# Autodesk Inventor assembly: Filament_dryer
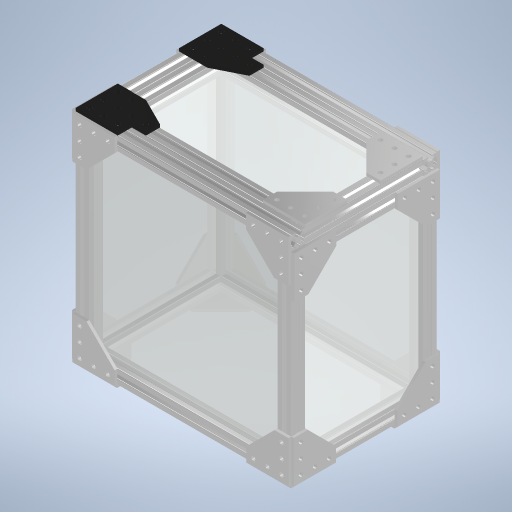
[picture p0: Inventor's stored thumbnail of the model, 512x512]
Saved by Autodesk Inventor 2024 (Build 280153000, 153)
## iProperties
Created: 2024-09-20
Part Number: Filament_dryer
Document SubType Name: Assembly
Designer: Owner
Author: Owner
## Documents named in this file (12)
- C:\Users\Owner\Desktop\Work\Filament dryer\Filament_dryer.iam
- C:\Users\Owner\Desktop\Work\Filament dryer\panel_14x9.ipt
- C:\Users\Owner\Desktop\Work\Filament dryer\T_slot_1in_8.35in.ipt
- C:\Users\Owner\Desktop\Work\Filament dryer\T_slot_1in_15.35in.ipt
- C:\Users\Owner\Desktop\Work\Filament dryer\panel_14x14.ipt
- C:\Users\Owner\Desktop\Work\Filament dryer\T_slot_1in_13.35in.ipt
- C:\Users\Owner\Desktop\Work\Filament dryer\panel_13x7.ipt
- C:\Users\Owner\Desktop\Work\Filament dryer\T_slot_1in_12.35in.ipt
- C:\Users\Owner\Desktop\Work\Filament dryer\panel_13x9.ipt
- C:\Users\Owner\Desktop\Work\Filament dryer\corner_bracket.ipt
- C:\Users\Owner\Desktop\Work\Filament dryer\47065T267_T-Slotted Framing_cut.ipt
- C:\Users\Owner\Desktop\Work\Filament dryer\corner_bracket_flush.ipt
## Components (48 placed, 11 different names)
1. panel_14x9:1 — Mate:1, Tangent:1, Flush:1, Mate:2, Flush:2, Tangent:2, Mate:3, Mate:4
2. T_slot_1in_8.35in:1 — Mate:2, Flush:2, Tangent:2, Mate:17, Flush:58, Flush:61, Flush:67, Flush:69
3. T_slot_1in_8.35in:2 — Mate:1, Tangent:1, Flush:1, Flush:3, Flush:4, Flush:5, Flush:6, Mate:32, Mate:40, Flush:35, Flush:36, Flush:63, Flush:64
4. T_slot_1in_15.35in:1 — Mate:3, Flush:3, Flush:4, Mate:5, Tangent:3, Flush:7, Mate:10, Mate:38, Flush:31, Mate:39, Flush:33, Mate:52, Mate:55, Flush:65, Mate:57, Flush:68
5. T_slot_1in_15.35in:2 — Mate:4, Flush:5, Flush:6, Mate:6, Tangent:4, Flush:8, Mate:12, Mate:16, Mate:41, Mate:50, Flush:54, Mate:51, Flush:57, Mate:53, Mate:54, Flush:62, Mate:56, Flush:66
6. panel_14x14:1 — Mate:5, Tangent:3, Flush:7, Mate:7, Tangent:5, Flush:9, Mate:9, Mate:13
7. panel_14x14:2 — Mate:6, Tangent:4, Flush:8, Mate:8, Tangent:6, Flush:10, Mate:11, Mate:15
8. T_slot_1in_15.35in:3 — Mate:8, Tangent:6, Flush:10, Flush:12, Flush:14, Mate:20, Flush:15, Mate:24, Mate:29, Flush:21, Flush:38, Mate:48, Mate:49, Flush:52, Flush:75
9. T_slot_1in_15.35in:4 — Mate:7, Tangent:5, Flush:9, Flush:11, Mate:14, Flush:13, Mate:23, Flush:18, Mate:27, Flush:20, Mate:34, Flush:22, Mate:35, Flush:24, Flush:25, Mate:47, Mate:61, Flush:77
10. T_slot_1in_13.35in:1 — Mate:15, Flush:14, Mate:16, Mate:21, Flush:16, Flush:17, Mate:33, Tangent:9, Mate:37, Flush:29, Flush:37, Mate:42, Flush:39, Flush:56
11. T_slot_1in_13.35in:2 — Mate:13, Mate:14, Flush:13, Mate:36, Flush:26, Flush:32, Flush:34
12. T_slot_1in_13.35in:3 — Mate:11, Flush:12, Mate:12, Flush:51, Flush:53, Flush:55, Flush:60
13. T_slot_1in_13.35in:4 — Mate:9, Flush:11, Mate:10, Mate:18, Tangent:7, Flush:23, Flush:30, Flush:49, Flush:59
14. panel_14x9:2 — Mate:17, Mate:18, Tangent:7, Mate:19
15. T_slot_1in_8.35in:3 — Mate:19, Mate:20, Flush:15, Flush:19, Mate:25, Flush:48, Flush:50, Mate:60, Flush:74, Flush:76
16. T_slot_1in_8.35in:4 — Mate:22, Mate:23, Flush:18, Mate:43, Flush:41, Mate:44, Flush:43
17. T_slot_1in_8.35in:5 — Mate:21, Flush:16, Flush:17, Mate:22, Flush:27, Flush:28
18. T_slot_1in_8.35in:6 — Mate:24, Flush:19, Mate:25, Mate:26, Mate:28, Mate:30, Flush:71, Mate:59, Flush:73
19. T_slot_1in_12.35in:1 — Mate:28, Mate:29, Flush:21, Mate:31, Tangent:8, Flush:42, Flush:72
20. T_slot_1in_12.35in:2 — Mate:26, Mate:27, Flush:20, Flush:40, Mate:58, Flush:70
21. panel_13x7:1 — Mate:30, Mate:31, Tangent:8
22. panel_13x9:1 — Mate:32, Mate:33, Tangent:9
23. corner_bracket:1 — Mate:39, Flush:32, Flush:33
24. corner_bracket:2 — Mate:40, Flush:34, Flush:35
25. corner_bracket:3 — Mate:42, Flush:38, Flush:39
26. corner_bracket:4 — Mate:43, Flush:40, Flush:41
27. corner_bracket:5 — Mate:38, Flush:30, Flush:31
28. corner_bracket:6 — Mate:34, Flush:22, Flush:23
29. corner_bracket:7 — Mate:41, Flush:36, Flush:37
30. corner_bracket:8 — Mate:35, Flush:24, Flush:25
31. corner_bracket:9 — Mate:37, Flush:28, Flush:29
32. corner_bracket:10 — Mate:36, Flush:26, Flush:27
33. corner_bracket:11 — Mate:51, Flush:56, Flush:57
34. corner_bracket:12 — Mate:44, Flush:42, Flush:43
35. corner_bracket:14 — Mate:52, Flush:58, Flush:59
36. corner_bracket:15 — Mate:53, Flush:60, Flush:61
37. corner_bracket:16 — Mate:48, Flush:50, Flush:51
38. corner_bracket:18 — Mate:50, Flush:54, Flush:55
39. corner_bracket:19 — Mate:49, Flush:52, Flush:53
40. corner_bracket:20 — Mate:47, Flush:48, Flush:49
41. corner_bracket:21 — Mate:55, Flush:64, Flush:65
42. corner_bracket:22 — Mate:57, Flush:68, Flush:69
43. corner_bracket:23 — Mate:56, Flush:66, Flush:67
44. corner_bracket:24 — Mate:54, Flush:62, Flush:63
45. 47065T267_T-Slotted Framing_cut:1 — Mate:59, Flush:72, Flush:73
46. 47065T267_T-Slotted Framing_cut:2 — Mate:58, Flush:70, Flush:71
47. corner_bracket_flush:1 — Mate:60, Flush:74, Flush:75
48. corner_bracket_flush:2 — Mate:61, Flush:76, Flush:77
## Relationships (141: Flush 73, Mate 59, Tangent 9)
- Mate:1: panel_14x9:1 ↔ T_slot_1in_8.35in:2
- Tangent:1: panel_14x9:1 ↔ T_slot_1in_8.35in:2
- Flush:1 (8.255 mm): panel_14x9:1 ↔ T_slot_1in_8.35in:2
- Mate:2: panel_14x9:1 ↔ T_slot_1in_8.35in:1
- Flush:2 (8.255 mm): panel_14x9:1 ↔ T_slot_1in_8.35in:1
- Tangent:2: panel_14x9:1 ↔ T_slot_1in_8.35in:1
- Mate:3: panel_14x9:1 ↔ T_slot_1in_15.35in:1
- Flush:3: T_slot_1in_8.35in:2 ↔ T_slot_1in_15.35in:1
- Flush:4: T_slot_1in_8.35in:2 ↔ T_slot_1in_15.35in:1
- Mate:4: panel_14x9:1 ↔ T_slot_1in_15.35in:2
- Flush:5: T_slot_1in_8.35in:2 ↔ T_slot_1in_15.35in:2
- Flush:6: T_slot_1in_8.35in:2 ↔ T_slot_1in_15.35in:2
- Mate:5: T_slot_1in_15.35in:1 ↔ panel_14x14:1
- Tangent:3: T_slot_1in_15.35in:1 ↔ panel_14x14:1
- Flush:7 (16.51 mm): T_slot_1in_15.35in:1 ↔ panel_14x14:1
- Mate:6: T_slot_1in_15.35in:2 ↔ panel_14x14:2
- Tangent:4: T_slot_1in_15.35in:2 ↔ panel_14x14:2
- Flush:8 (16.51 mm): T_slot_1in_15.35in:2 ↔ panel_14x14:2
- Mate:7: panel_14x14:1 ↔ T_slot_1in_15.35in:4
- Tangent:5: panel_14x14:1 ↔ T_slot_1in_15.35in:4
- Flush:9 (-16.51 mm): panel_14x14:1 ↔ T_slot_1in_15.35in:4
- Mate:8: panel_14x14:2 ↔ T_slot_1in_15.35in:3
- Tangent:6: panel_14x14:2 ↔ T_slot_1in_15.35in:3
- Flush:10 (-16.51 mm): panel_14x14:2 ↔ T_slot_1in_15.35in:3
- Mate:9: panel_14x14:1 ↔ T_slot_1in_13.35in:4
- Flush:11: T_slot_1in_15.35in:4 ↔ T_slot_1in_13.35in:4
- Mate:10: T_slot_1in_15.35in:1 ↔ T_slot_1in_13.35in:4
- Mate:11: panel_14x14:2 ↔ T_slot_1in_13.35in:3
- Flush:12: T_slot_1in_15.35in:3 ↔ T_slot_1in_13.35in:3
- Mate:12: T_slot_1in_15.35in:2 ↔ T_slot_1in_13.35in:3
- Mate:13: panel_14x14:1 ↔ T_slot_1in_13.35in:2
- Mate:14: T_slot_1in_15.35in:4 ↔ T_slot_1in_13.35in:2
- Flush:13: T_slot_1in_15.35in:4 ↔ T_slot_1in_13.35in:2
- Mate:15: panel_14x14:2 ↔ T_slot_1in_13.35in:1
- Flush:14: T_slot_1in_15.35in:3 ↔ T_slot_1in_13.35in:1
- Mate:16: T_slot_1in_15.35in:2 ↔ T_slot_1in_13.35in:1
- Mate:17: T_slot_1in_8.35in:1 ↔ panel_14x9:2
- Mate:18: T_slot_1in_13.35in:4 ↔ panel_14x9:2
- Tangent:7: T_slot_1in_13.35in:4 ↔ panel_14x9:2
- Mate:19: panel_14x9:2 ↔ T_slot_1in_8.35in:3
- Mate:20: T_slot_1in_15.35in:3 ↔ T_slot_1in_8.35in:3
- Flush:15: T_slot_1in_15.35in:3 ↔ T_slot_1in_8.35in:3
- Mate:21: T_slot_1in_13.35in:1 ↔ T_slot_1in_8.35in:5
- Flush:16: T_slot_1in_13.35in:1 ↔ T_slot_1in_8.35in:5
- Flush:17: T_slot_1in_13.35in:1 ↔ T_slot_1in_8.35in:5
- Mate:22: T_slot_1in_8.35in:4 ↔ T_slot_1in_8.35in:5
- Mate:23: T_slot_1in_15.35in:4 ↔ T_slot_1in_8.35in:4
- Flush:18: T_slot_1in_15.35in:4 ↔ T_slot_1in_8.35in:4
- Mate:24: T_slot_1in_15.35in:3 ↔ T_slot_1in_8.35in:6
- Flush:19: T_slot_1in_8.35in:3 ↔ T_slot_1in_8.35in:6
- Mate:25: T_slot_1in_8.35in:3 ↔ T_slot_1in_8.35in:6
- Mate:26: T_slot_1in_8.35in:6 ↔ T_slot_1in_12.35in:2
- Mate:27: T_slot_1in_15.35in:4 ↔ T_slot_1in_12.35in:2
- Flush:20: T_slot_1in_15.35in:4 ↔ T_slot_1in_12.35in:2
- Mate:28: T_slot_1in_8.35in:6 ↔ T_slot_1in_12.35in:1
- Mate:29: T_slot_1in_15.35in:3 ↔ T_slot_1in_12.35in:1
- Flush:21: T_slot_1in_15.35in:3 ↔ T_slot_1in_12.35in:1
- Mate:30: T_slot_1in_8.35in:6 ↔ panel_13x7:1
- Mate:31: T_slot_1in_12.35in:1 ↔ panel_13x7:1
- Tangent:8: T_slot_1in_12.35in:1 ↔ panel_13x7:1
- Mate:32: T_slot_1in_8.35in:2 ↔ panel_13x9:1
- Mate:33: T_slot_1in_13.35in:1 ↔ panel_13x9:1
- Tangent:9: T_slot_1in_13.35in:1 ↔ panel_13x9:1
- Mate:34: T_slot_1in_15.35in:4 ↔ corner_bracket:6
- Flush:22: T_slot_1in_15.35in:4 ↔ corner_bracket:6
- Flush:23: T_slot_1in_13.35in:4 ↔ corner_bracket:6
- Mate:35: T_slot_1in_15.35in:4 ↔ corner_bracket:8
- Flush:24: T_slot_1in_15.35in:4 ↔ corner_bracket:8
- Flush:25: T_slot_1in_15.35in:4 ↔ corner_bracket:8
- Mate:36: T_slot_1in_13.35in:2 ↔ corner_bracket:10
- Flush:26: T_slot_1in_13.35in:2 ↔ corner_bracket:10
- Flush:27: T_slot_1in_8.35in:5 ↔ corner_bracket:10
- Mate:37: T_slot_1in_13.35in:1 ↔ corner_bracket:9
- Flush:28: T_slot_1in_8.35in:5 ↔ corner_bracket:9
- Flush:29: T_slot_1in_13.35in:1 ↔ corner_bracket:9
- Mate:38: T_slot_1in_15.35in:1 ↔ corner_bracket:5
- Flush:30: T_slot_1in_13.35in:4 ↔ corner_bracket:5
- Flush:31: T_slot_1in_15.35in:1 ↔ corner_bracket:5
- Mate:39: T_slot_1in_15.35in:1 ↔ corner_bracket:1
- Flush:32: T_slot_1in_13.35in:2 ↔ corner_bracket:1
- Flush:33: T_slot_1in_15.35in:1 ↔ corner_bracket:1
- Mate:40: T_slot_1in_8.35in:2 ↔ corner_bracket:2
- Flush:34: T_slot_1in_13.35in:2 ↔ corner_bracket:2
- Flush:35: T_slot_1in_8.35in:2 ↔ corner_bracket:2
- Mate:41: T_slot_1in_15.35in:2 ↔ corner_bracket:7
- Flush:36: T_slot_1in_8.35in:2 ↔ corner_bracket:7
- Flush:37: T_slot_1in_13.35in:1 ↔ corner_bracket:7
- Mate:42: T_slot_1in_13.35in:1 ↔ corner_bracket:3
- Flush:38: T_slot_1in_15.35in:3 ↔ corner_bracket:3
- Flush:39: T_slot_1in_13.35in:1 ↔ corner_bracket:3
- Mate:43: T_slot_1in_8.35in:4 ↔ corner_bracket:4
- Flush:40: T_slot_1in_12.35in:2 ↔ corner_bracket:4
- Flush:41: T_slot_1in_8.35in:4 ↔ corner_bracket:4
- Mate:44: T_slot_1in_8.35in:4 ↔ corner_bracket:12
- Flush:42: T_slot_1in_12.35in:1 ↔ corner_bracket:12
- Flush:43: T_slot_1in_8.35in:4 ↔ corner_bracket:12
- Mate:47: T_slot_1in_15.35in:4 ↔ corner_bracket:20
- Flush:48: T_slot_1in_8.35in:3 ↔ corner_bracket:20
- Flush:49: T_slot_1in_13.35in:4 ↔ corner_bracket:20
- Mate:48: T_slot_1in_15.35in:3 ↔ corner_bracket:16
- Flush:50: T_slot_1in_8.35in:3 ↔ corner_bracket:16
- Flush:51: T_slot_1in_13.35in:3 ↔ corner_bracket:16
- Mate:49: T_slot_1in_15.35in:3 ↔ corner_bracket:19
- Flush:52: T_slot_1in_15.35in:3 ↔ corner_bracket:19
- Flush:53: T_slot_1in_13.35in:3 ↔ corner_bracket:19
- Mate:50: T_slot_1in_15.35in:2 ↔ corner_bracket:18
- Flush:54: T_slot_1in_15.35in:2 ↔ corner_bracket:18
- Flush:55: T_slot_1in_13.35in:3 ↔ corner_bracket:18
- Mate:51: T_slot_1in_15.35in:2 ↔ corner_bracket:11
- Flush:56: T_slot_1in_13.35in:1 ↔ corner_bracket:11
- Flush:57: T_slot_1in_15.35in:2 ↔ corner_bracket:11
- Mate:52: T_slot_1in_15.35in:1 ↔ corner_bracket:14
- Flush:58: T_slot_1in_8.35in:1 ↔ corner_bracket:14
- Flush:59: T_slot_1in_13.35in:4 ↔ corner_bracket:14
- Mate:53: T_slot_1in_15.35in:2 ↔ corner_bracket:15
- Flush:60: T_slot_1in_13.35in:3 ↔ corner_bracket:15
- Flush:61: T_slot_1in_8.35in:1 ↔ corner_bracket:15
- Mate:54: T_slot_1in_15.35in:2 ↔ corner_bracket:24
- Flush:62: T_slot_1in_15.35in:2 ↔ corner_bracket:24
- Flush:63: T_slot_1in_8.35in:2 ↔ corner_bracket:24
- Mate:55: T_slot_1in_15.35in:1 ↔ corner_bracket:21
- Flush:64: T_slot_1in_8.35in:2 ↔ corner_bracket:21
- Flush:65: T_slot_1in_15.35in:1 ↔ corner_bracket:21
- Mate:56: T_slot_1in_15.35in:2 ↔ corner_bracket:23
- Flush:66: T_slot_1in_15.35in:2 ↔ corner_bracket:23
- Flush:67: T_slot_1in_8.35in:1 ↔ corner_bracket:23
- Mate:57: T_slot_1in_15.35in:1 ↔ corner_bracket:22
- Flush:68: T_slot_1in_15.35in:1 ↔ corner_bracket:22
- Flush:69: T_slot_1in_8.35in:1 ↔ corner_bracket:22
- Mate:58: T_slot_1in_12.35in:2 ↔ 47065T267_T-Slotted Framing_cut:2
- Flush:70: T_slot_1in_12.35in:2 ↔ 47065T267_T-Slotted Framing_cut:2
- Flush:71: T_slot_1in_8.35in:6 ↔ 47065T267_T-Slotted Framing_cut:2
- Mate:59: T_slot_1in_8.35in:6 ↔ 47065T267_T-Slotted Framing_cut:1
- Flush:72: T_slot_1in_12.35in:1 ↔ 47065T267_T-Slotted Framing_cut:1
- Flush:73: T_slot_1in_8.35in:6 ↔ 47065T267_T-Slotted Framing_cut:1
- Mate:60: T_slot_1in_8.35in:3 ↔ corner_bracket_flush:1
- Flush:74: T_slot_1in_8.35in:3 ↔ corner_bracket_flush:1
- Flush:75: T_slot_1in_15.35in:3 ↔ corner_bracket_flush:1
- Mate:61: T_slot_1in_15.35in:4 ↔ corner_bracket_flush:2
- Flush:76: T_slot_1in_8.35in:3 ↔ corner_bracket_flush:2
- Flush:77: T_slot_1in_15.35in:4 ↔ corner_bracket_flush:2
